# Autodesk Inventor assembly: 100-10-FRAME-TOP-01
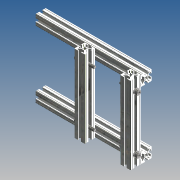
[picture p0: Inventor's stored thumbnail of the model, 180x180]
Saved by Autodesk Inventor 2018.2 (Build 222227000, 227)
## iProperties
Manager: feesmrt
Company: FRANCOR
Part Number: 100-10-FRAME-TOP-01
Project: Rescue Robot
Cost Center: -
Material: Generisch
Document SubType Name: Assembly
Designer: feesmrt
Engineer: feesmrt
Authority: feesmrt
Subject: Rescue Robot
Author: feesmrt
Revision Number: 1
## Documents named in this file (5)
- C:\Users\feesmrt\Documents\FRANC0R\CAD\02-Rocker-Bogie-Robot\100-CHASSIS\10-FRAME\100-10-FRAME-TOP-01.iam
- C:\Users\feesmrt\Documents\FRANC0R\CAD\02-Rocker-Bogie-Robot\100-CHASSIS\10-FRAME\100-10-FRAME-PROFILE-ROCKER-CONNECTOR.ipt
- C:\Users\feesmrt\Documents\FRANC0R\CAD\02-Rocker-Bogie-Robot\100-CHASSIS\10-FRAME\100-10-FRAME-ROCKER-SCREW-01.iam
- C:\Users\feesmrt\Documents\FRANC0R\CAD\02-Rocker-Bogie-Robot\100-CHASSIS\10-FRAME\100-10-FRAME-PROFILE-TOP-L-01.ipt
- C:\Users\feesmrt\Documents\FRANC0R\CAD\02-Rocker-Bogie-Robot\100-CHASSIS\Chassis-Dimensions.xlsx
## Components (8 placed, 3 different names)
1. 100-10-FRAME-PROFILE-ROCKER-CONNECTOR:1 — Fluchtend:1, Passend:2, Passend:5, Passend:6, Passend:7, Passend:8, Fluchtend:4, Passend:13, Fluchtend:5, Fluchtend:6
2. 100-10-FRAME-PROFILE-ROCKER-CONNECTOR:2 — Fluchtend:2, Passend:1, Passend:2, Passend:3, Passend:4, Passend:9, Passend:10, Passend:12, Fluchtend:3
3. 100-10-FRAME-ROCKER-SCREW-01:1 [sub-assembly] — Passend:5, Passend:8
4. 100-10-FRAME-ROCKER-SCREW-01:2 [sub-assembly] — Passend:6, Passend:7
5. 100-10-FRAME-ROCKER-SCREW-01:3 [sub-assembly] — Passend:3, Passend:9
6. 100-10-FRAME-ROCKER-SCREW-01:4 [sub-assembly] — Passend:4, Passend:10
7. 100-10-FRAME-PROFILE-TOP-L-01:1 — Passend:12, Fluchtend:3, Fluchtend:4
8. 100-10-FRAME-PROFILE-TOP-L-01:2 — Passend:13, Fluchtend:5, Fluchtend:6
## Relationships (18: Mate 12, Flush 6)
- Fluchtend:1 [Flush]: 100-10-FRAME-PROFILE-ROCKER-CONNECTOR:1
- Fluchtend:2 [Flush]: 100-10-FRAME-PROFILE-ROCKER-CONNECTOR:2
- Passend:1 [Mate]: 100-10-FRAME-PROFILE-ROCKER-CONNECTOR:2
- Passend:2 [Mate] (100 mm): 100-10-FRAME-PROFILE-ROCKER-CONNECTOR:1 ↔ 100-10-FRAME-PROFILE-ROCKER-CONNECTOR:2
- Passend:3 [Mate]: 100-10-FRAME-PROFILE-ROCKER-CONNECTOR:2 ↔ 100-10-FRAME-ROCKER-SCREW-01:3
- Passend:4 [Mate]: 100-10-FRAME-PROFILE-ROCKER-CONNECTOR:2 ↔ 100-10-FRAME-ROCKER-SCREW-01:4
- Passend:5 [Mate]: 100-10-FRAME-PROFILE-ROCKER-CONNECTOR:1 ↔ 100-10-FRAME-ROCKER-SCREW-01:1
- Passend:6 [Mate]: 100-10-FRAME-PROFILE-ROCKER-CONNECTOR:1 ↔ 100-10-FRAME-ROCKER-SCREW-01:2
- Passend:7 [Mate]: 100-10-FRAME-PROFILE-ROCKER-CONNECTOR:1 ↔ 100-10-FRAME-ROCKER-SCREW-01:2
- Passend:8 [Mate]: 100-10-FRAME-PROFILE-ROCKER-CONNECTOR:1 ↔ 100-10-FRAME-ROCKER-SCREW-01:1
- Passend:9 [Mate]: 100-10-FRAME-PROFILE-ROCKER-CONNECTOR:2 ↔ 100-10-FRAME-ROCKER-SCREW-01:3
- Passend:10 [Mate]: 100-10-FRAME-PROFILE-ROCKER-CONNECTOR:2 ↔ 100-10-FRAME-ROCKER-SCREW-01:4
- Passend:12 [Mate]: 100-10-FRAME-PROFILE-ROCKER-CONNECTOR:2 ↔ 100-10-FRAME-PROFILE-TOP-L-01:1
- Fluchtend:3 [Flush]: 100-10-FRAME-PROFILE-ROCKER-CONNECTOR:2 ↔ 100-10-FRAME-PROFILE-TOP-L-01:1
- Fluchtend:4 [Flush]: 100-10-FRAME-PROFILE-ROCKER-CONNECTOR:1 ↔ 100-10-FRAME-PROFILE-TOP-L-01:1
- Passend:13 [Mate]: 100-10-FRAME-PROFILE-ROCKER-CONNECTOR:1 ↔ 100-10-FRAME-PROFILE-TOP-L-01:2
- Fluchtend:5 [Flush]: 100-10-FRAME-PROFILE-ROCKER-CONNECTOR:1 ↔ 100-10-FRAME-PROFILE-TOP-L-01:2
- Fluchtend:6 [Flush]: 100-10-FRAME-PROFILE-ROCKER-CONNECTOR:1 ↔ 100-10-FRAME-PROFILE-TOP-L-01:2
## Named parameters: Chassis_Frame_Size = 30 mm, Chassis_Length = 500 mm, Chassis_Width = 220 mm, Rocker_Bearing_Size = 100 mm, Rocker_Screw_Distance = 32.5 mm, Rocker_Screw_Distance_Bottom = 76 mm, Chassis_Bottom_Height = 80 mm
